# Autodesk Inventor assembly: ASY составное колено из труб
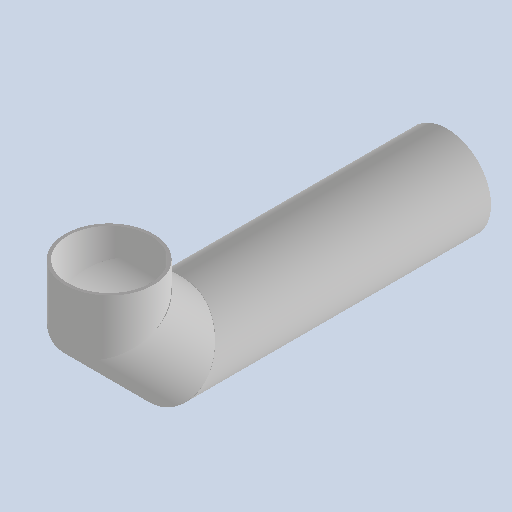
[picture p0: Inventor's stored thumbnail of the model, 512x512]
Saved by Autodesk Inventor 2024.2 (Build 282272000, 272)
## iProperties
Created: 2024-06-07
Part Number: ASY составное колено из труб
Document SubType Name: Assembly
Designer: admin
Author: admin
## Documents named in this file (4)
- C:\Users\admin\YandexDisk-badmisterfox\домашниий пк\Inventor\Manturovo\Manturovo_Se-clar\ASY составное колено из труб.iam
- C:\Users\admin\YandexDisk-badmisterfox\домашниий пк\Inventor\Manturovo\Manturovo_Se-clar\ракета\МОО 065 ракета труба 5.ipt
- C:\Users\admin\YandexDisk-badmisterfox\домашниий пк\Inventor\Manturovo\Manturovo_Se-clar\ракета\МОО 066 ракета труба 6.ipt
- C:\Users\admin\YandexDisk-badmisterfox\домашниий пк\Inventor\Manturovo\Manturovo_Se-clar\ракета\МОО 067 ракета труба 7.ipt
## Components (3 placed, 3 different names)
1. МОО 065 ракета труба 5:1
2. МОО 066 ракета труба 6:1
3. МОО 067 ракета труба 7:1
## Relationships (2: WeldJoint 2)
- [WeldJoint]: МОО 065 ракета труба 5:1 ↔ МОО 066 ракета труба 6:1
- [WeldJoint]: МОО 066 ракета труба 6:1 ↔ МОО 067 ракета труба 7:1
